# Autodesk Inventor assembly: Assembly
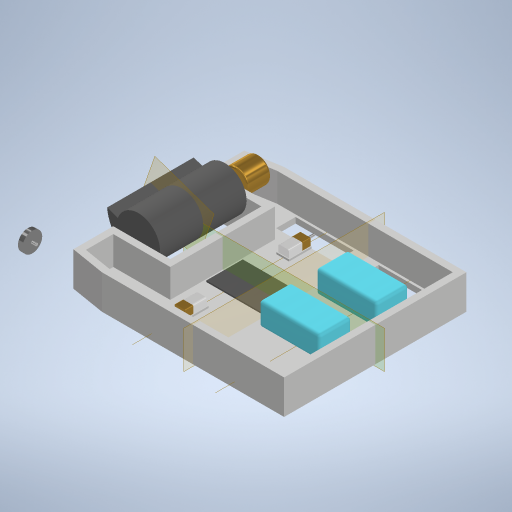
[picture p0: Inventor's stored thumbnail of the model, 512x512]
Saved by Autodesk Inventor 2024 (Build 280153000, 153)
## iProperties
Created: 2023-10-18
Part Number: Assembly
Document SubType Name: Assembly
Designer: CJ110
Author: CJ110
## Documents named in this file (8)
- D:\GitHub\Vault-1\CAD\WCRL\V1\Bot Assembly.iam
- D:\GitHub\Vault-1\CAD\WCRL\V1\Bot v1 bottom.ipt
- D:\GitHub\Vault-1\CAD\WCRL\V1\DC 6V 200RPM.ipt
- D:\GitHub\Vault-1\CAD\WCRL\V1\Brushless 2826 2200KV.ipt
- D:\GitHub\Vault-1\CAD\WCRL\V1\Brushless 2205 2300KV.ipt
- D:\GitHub\Vault-1\CAD\WCRL\V1\PCB.ipt
- D:\GitHub\Vault-1\CAD\WCRL\V1\LiPo.ipt
- D:\GitHub\Vault-1\CAD\WCRL\V1\Drum.ipt
## Components (9 placed, 7 different names)
1. Bot v1 bottom:1 — Mate:1, Mate:2, Mate:4, Mate:5, Mate:6, Mate:7, Mate:8, Mate:9, Mate:11, Mate:12, Mate:13, Mate:14, Mate:15
2. DC 6V 200RPM:1 — Mate:2, Mate:14, Mate:15
3. DC 6V 200RPM:2 — Mate:1, Mate:12, Mate:13
4. Brushless 2826 2200KV:1 — Mate:8, Mate:9, Mate:10
5. Brushless 2205 2300KV:1 — Mate:4
6. PCB:1 — Mate:5
7. LiPo:1 — Mate:7
8. LiPo:2 — Mate:6
9. Drum:1 — Mate:10, Mate:11
## Relationships (14: Mate 14)
- Mate:1: Bot v1 bottom:1 ↔ DC 6V 200RPM:2
- Mate:2: Bot v1 bottom:1 ↔ DC 6V 200RPM:1
- Mate:4: Bot v1 bottom:1 ↔ Brushless 2205 2300KV:1
- Mate:5: Bot v1 bottom:1 ↔ PCB:1
- Mate:6: Bot v1 bottom:1 ↔ LiPo:2
- Mate:7: Bot v1 bottom:1 ↔ LiPo:1
- Mate:8: Bot v1 bottom:1 ↔ Brushless 2826 2200KV:1
- Mate:9 (1.27 mm): Bot v1 bottom:1 ↔ Brushless 2826 2200KV:1
- Mate:10: Brushless 2826 2200KV:1 ↔ Drum:1
- Mate:11: Bot v1 bottom:1 ↔ Drum:1
- Mate:12: Bot v1 bottom:1 ↔ DC 6V 200RPM:2
- Mate:13: Bot v1 bottom:1 ↔ DC 6V 200RPM:2
- Mate:14: Bot v1 bottom:1 ↔ DC 6V 200RPM:1
- Mate:15: Bot v1 bottom:1 ↔ DC 6V 200RPM:1
